# Autodesk Inventor assembly: CollectionProto
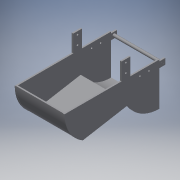
[picture p0: Inventor's stored thumbnail of the model, 180x180]
Saved by Autodesk Inventor 2019 (Build 230136000, 136)
## iProperties
Created: 2018-10-04
Part Number: CollectionProto
Document SubType Name: Assembly
Designer: User
Author: User
## Documents named in this file (5)
- C:\Robotics\CAD\2018-19_CAD\Collection\CollectionProto.iam
- C:\Robotics\CAD\2018-19_CAD\Collection\CollectorFloor.ipt
- C:\Robotics\CAD\2018-19_CAD\Collection\CollectorSweeperBacking.ipt
- C:\Robotics\CAD\2018-19_CAD\Collection\CollectionCasing.ipt
- C:\Robotics\CAD\2018-19_CAD\Collection\4inAxle.ipt
## Components (6 placed, 4 different names)
1. CollectorFloor:1 — Mate:2, Mate:3, Angle:1, Angle:2, Flush:1, Flush:2, Angle:3, Mate:5
2. CollectorSweeperBacking:1 — Mate:3, Angle:2, Flush:2, Flush:4, Flush:5
3. CollectorSweeperBacking:2 — Mate:2, Angle:1, Flush:1, Mate:1, Mate:4, Flush:3, Flush:6
4. CollectionCasing:1 — Mate:4, Flush:3, Flush:4, Mate:6, Insert:1
5. CollectionCasing:2 — Flush:5, Flush:6, Mate:5
6. 4inAxle:1 — Insert:1
## Relationships (16: Mate 6, Flush 6, Angle 3, Insert 1)
- Mate:1: CollectorSweeperBacking:2
- Mate:2: CollectorFloor:1 ↔ CollectorSweeperBacking:2
- Mate:3: CollectorFloor:1 ↔ CollectorSweeperBacking:1
- Angle:1 (-10 deg): CollectorFloor:1 ↔ CollectorSweeperBacking:2
- Angle:2 (100 deg): CollectorFloor:1 ↔ CollectorSweeperBacking:1
- Flush:1: CollectorFloor:1 ↔ CollectorSweeperBacking:2
- Flush:2: CollectorFloor:1 ↔ CollectorSweeperBacking:1
- Angle:3 (-10 deg): CollectorFloor:1
- Mate:4: CollectorSweeperBacking:2 ↔ CollectionCasing:1
- Flush:3: CollectorSweeperBacking:2 ↔ CollectionCasing:1
- Flush:4: CollectorSweeperBacking:1 ↔ CollectionCasing:1
- Flush:5: CollectorSweeperBacking:1 ↔ CollectionCasing:2
- Flush:6: CollectorSweeperBacking:2 ↔ CollectionCasing:2
- Mate:5: CollectorFloor:1 ↔ CollectionCasing:2
- Mate:6: CollectionCasing:1
- Insert:1: CollectionCasing:1 ↔ 4inAxle:1
